# Autodesk Inventor assembly: ServoAssemblyActual
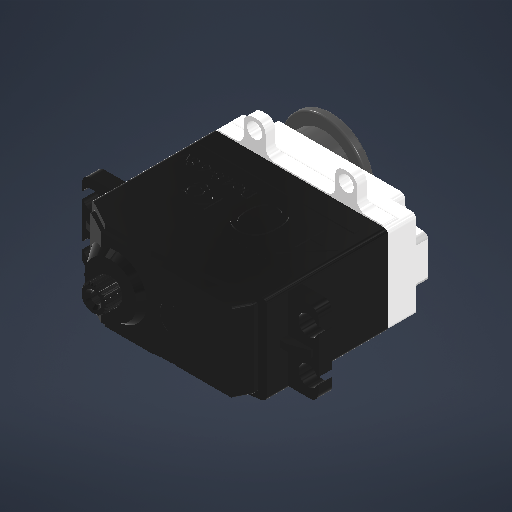
[picture p0: Inventor's stored thumbnail of the model, 512x512]
Saved by Autodesk Inventor 2026.2 (Build 302298010, 298A)
## iProperties
Created: 2026-03-14
Part Number: ServoAssemblyActual
Document SubType Name: Assembly
Designer: Liam
Author: Liam
## Documents named in this file (4)
- C:\Users\Liam\OneDrive\Documents\Inventor\Hexapod\V2\ServoAssemblyActual.iam
- C:\Users\Liam\OneDrive\Documents\Inventor\Hexapod\DS3240NoBottom.ipt
- C:\Users\Liam\OneDrive\Documents\Inventor\Hexapod\V2\ServoCase10mmSideExit.ipt
- C:\Users\Liam\OneDrive\Documents\Inventor\Hexapod\V2\AxleCap.ipt
## Components (3 placed, 3 different names)
1. DS3240NoBottom:1 — Rigid:1
2. ServoCase10mmSideExit:1 — Rigid:1, Rigid:2
3. AxleCap:1 — Rigid:2
## Relationships (2: WeldJoint 2)
- Rigid:1 [WeldJoint]: DS3240NoBottom:1 ↔ ServoCase10mmSideExit:1
- Rigid:2 [WeldJoint]: ServoCase10mmSideExit:1 ↔ AxleCap:1
